# Autodesk Inventor assembly: Assembly23
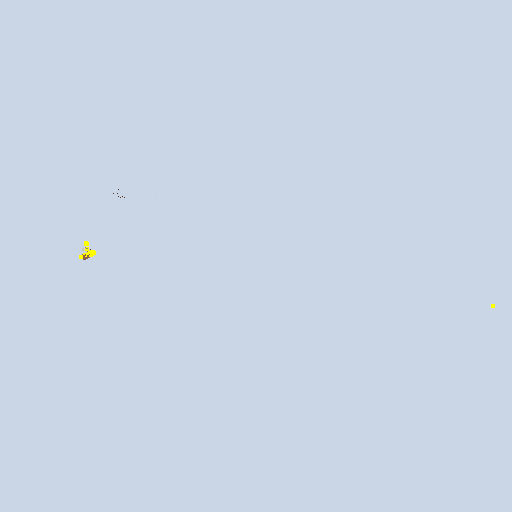
[picture p0: Inventor's stored thumbnail of the model, 512x512]
Saved by Autodesk Inventor 2024.1 (Build 281209000, 209)
## iProperties
Created: 2023-11-10
Part Number: Assembly23
Document SubType Name: Assembly
Designer: luvag
Author: luvag
## Documents named in this file (3)
- C:\Users\luvag\Desktop\Assembly23.iam
- C:\Users\luvag\Desktop\eg part 2.ipt
- C:\Users\luvag\Desktop\Assembly19.iam
## Components (3 placed, 2 different names)
1. eg part 2:1
2. eg part 2:2
3. Assembly19:1 [sub-assembly]
## Relationships (2: Mate 2)
- [Mate]: eg part 2:1 ↔ Assembly19:1
- [Mate]: eg part 2:2 ↔ Assembly19:1
